# Autodesk Inventor assembly: 0005-00-00 Ansamblu_General_V1
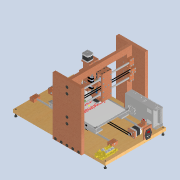
[picture p0: Inventor's stored thumbnail of the model, 180x180]
Saved by Autodesk Inventor 2020 (Build 240168000, 168)
## iProperties
Created: 2020-12-26
Part Number: 0005-00-00 Ansamblu_General_V1
Document SubType Name: Assembly
Designer: Iulian Bors
Author: Iulian Bors
## Documents named in this file (14)
- Z:\I.A.B\Proiecte\0005 I.A.B 3d 2.0 Imprimanta aracet\0005-00-00 Ansamblu_General_V1.iam
- Z:\I.A.B\Proiecte\0005 I.A.B 3d 2.0 Imprimanta aracet\10 Mecanic\0005-10-01 Cadru.iam
- Z:\I.A.B\Proiecte\0005 I.A.B 3d 2.0 Imprimanta aracet\10 Mecanic\0005-10-02 X axis.iam
- Z:\I.A.B\Proiecte\0005 I.A.B 3d 2.0 Imprimanta aracet\10 Mecanic\0005-10-03 Y axis.iam
- Z:\I.A.B\Proiecte\0005 I.A.B 3d 2.0 Imprimanta aracet\10 Mecanic\0005-10-04 Z axis and extruder.iam
- Z:\I.A.B\Proiecte\0005 I.A.B 3d 2.0 Imprimanta aracet\20 Electric\0005-20-01 Assembly Arduino Mega RAMPS 1.4.iam
- Z:\I.A.B\Proiecte\0005 I.A.B 3d 2.0 Imprimanta aracet\20 Electric\Inlet Module Plug Fuse Switch Male Power Socket 10A 250V 3 Pin IEC320 C14.ipt
- Z:\I.A.B\Proiecte\0005 I.A.B 3d 2.0 Imprimanta aracet\20 Electric\00005-20-1004 PowerSupplyLedMax500.ipt
- Z:\I.A.B\Proiecte\0005 I.A.B 3d 2.0 Imprimanta aracet\10 Mecanic\0005-10-1044 DIN EN ISO 1483 - ST3.5 x 13 - C.ipt
- Z:\I.A.B\Proiecte\0005 I.A.B 3d 2.0 Imprimanta aracet\20 Electric\0005-20-1003 Switch.ipt
- Z:\I.A.B\Proiecte\0005 I.A.B 3d 2.0 Imprimanta aracet\10 Mecanic\0005-10-028 suport senzor y.ipt
- Z:\I.A.B\Proiecte\0005 I.A.B 3d 2.0 Imprimanta aracet\10 Mecanic\0005-10-1032.ipt
- Z:\I.A.B\Proiecte\0005 I.A.B 3d 2.0 Imprimanta aracet\10 Mecanic\0005-10-1019 ISO 4762 - M3 x 30ISO.ipt
- Z:\I.A.B\Proiecte\0005 I.A.B 3d 2.0 Imprimanta aracet\10 Mecanic\0005-10-030 Activator senzor x.ipt
## Components (23 placed, 13 different names)
1. 0005-10-01 Cadru:1 [sub-assembly] — Insert:1, Mate:1, Mate:3, Flush:1, Flush:2, Mate:4, Flush:3, Flush:4, Mate:5, Mate:6, Mate:7, Mate:9, Mate:12, Mate:16, Mate:17, Insert:18, Insert:19, Mate:19, Flush:11
2. 0005-10-02 X axis:1 [sub-assembly] — Insert:1, Mate:1, Insert:2, Insert:3, Mate:18, Flush:10
3. 0005-10-03 Y axis:1 [sub-assembly] — Mate:3, Flush:1, Flush:2, Mate:11, Flush:5, Mate:13, Flush:6
4. 0005-10-04 Z axis and extruder:1 [sub-assembly] — Insert:2, Insert:3, Mate:15, Flush:8, Flush:9
5. 0005-20-01 Assembly Arduino Mega RAMPS 1.4:1 [sub-assembly] — Mate:4, Flush:3, Flush:4, Insert:15, Insert:16, Insert:17
6. Inlet Module Plug Fuse Switch Male Power Socket 10A 250V 3 Pin IEC320 C14:1 — Mate:5, Mate:6, Mate:7, Insert:4, Insert:5
7. 00005-20-1004 PowerSupplyLedMax500:1 — Mate:9, Mate:16, Mate:17
8. DIN EN ISO 1483 - C ST3.5 x 13 - C:1 — Insert:4
9. DIN EN ISO 1483 - C ST3.5 x 13 - C:2 — Insert:5
10. 0005-20-1003 Switch:1 — Mate:11, Mate:12, Flush:5, Insert:13, Insert:14
11. 0005-20-1003 Switch:2 — Mate:15, Flush:8, Flush:9, Insert:11, Insert:12
12. 0005-20-1003 Switch:3 — Mate:18, Flush:10
13. 0005-10-028 suport senzor y:1 — Mate:13, Flush:6
14. DIN 7984 M3 x 16:1 — Insert:14
15. DIN 7984 M3 x 16:2 — Insert:13
16. DIN 7984 M3 x 16:3 — Insert:12
17. DIN 7984 M3 x 16:4 — Insert:11
18. ISO 4762 M3 x 30:1 — Insert:15
19. ISO 4762 M3 x 30:2 — Insert:17
20. ISO 4762 M3 x 30:3 — Insert:16
21. ISO 4762 M3 x 30:4 — Insert:18
22. ISO 4762 M3 x 30:5 — Insert:19
23. 0005-10-030 Activator senzor x:1 — Mate:19, Flush:11
## Relationships (39: Mate 15, Insert 14, Flush 10)
- Insert:1: 0005-10-01 Cadru:1 ↔ 0005-10-02 X axis:1
- Mate:1: 0005-10-01 Cadru:1 ↔ 0005-10-02 X axis:1
- Mate:3: 0005-10-01 Cadru:1 ↔ 0005-10-03 Y axis:1
- Flush:1 (110 mm): 0005-10-01 Cadru:1 ↔ 0005-10-03 Y axis:1
- Flush:2 (5.193 mm): 0005-10-01 Cadru:1 ↔ 0005-10-03 Y axis:1
- Insert:2: 0005-10-02 X axis:1 ↔ 0005-10-04 Z axis and extruder:1
- Insert:3: 0005-10-02 X axis:1 ↔ 0005-10-04 Z axis and extruder:1
- Mate:4 (3 mm): 0005-10-01 Cadru:1 ↔ 0005-20-01 Assembly Arduino Mega RAMPS 1.4:1
- Flush:3 (-10 mm): 0005-10-01 Cadru:1 ↔ 0005-20-01 Assembly Arduino Mega RAMPS 1.4:1
- Flush:4 (20 mm): 0005-10-01 Cadru:1 ↔ 0005-20-01 Assembly Arduino Mega RAMPS 1.4:1
- Mate:5: 0005-10-01 Cadru:1 ↔ Inlet Module Plug Fuse Switch Male Power Socket 10A 250V 3 Pin IEC320 C14:1
- Mate:6: 0005-10-01 Cadru:1 ↔ Inlet Module Plug Fuse Switch Male Power Socket 10A 250V 3 Pin IEC320 C14:1
- Mate:7 (2 mm): 0005-10-01 Cadru:1 ↔ Inlet Module Plug Fuse Switch Male Power Socket 10A 250V 3 Pin IEC320 C14:1
- Mate:9: 0005-10-01 Cadru:1 ↔ 00005-20-1004 PowerSupplyLedMax500:1
- Insert:4: Inlet Module Plug Fuse Switch Male Power Socket 10A 250V 3 Pin IEC320 C14:1 ↔ DIN EN ISO 1483 - C ST3.5 x 13 - C:1
- Insert:5: Inlet Module Plug Fuse Switch Male Power Socket 10A 250V 3 Pin IEC320 C14:1 ↔ DIN EN ISO 1483 - C ST3.5 x 13 - C:2
- Mate:11 (8 mm): 0005-10-03 Y axis:1 ↔ 0005-20-1003 Switch:1
- Mate:12: 0005-10-01 Cadru:1 ↔ 0005-20-1003 Switch:1
- Flush:5: 0005-10-03 Y axis:1 ↔ 0005-20-1003 Switch:1
- Mate:13: 0005-10-03 Y axis:1 ↔ 0005-10-028 suport senzor y:1
- Flush:6: 0005-10-03 Y axis:1 ↔ 0005-10-028 suport senzor y:1
- Mate:15: 0005-10-04 Z axis and extruder:1 ↔ 0005-20-1003 Switch:2
- Flush:8: 0005-10-04 Z axis and extruder:1 ↔ 0005-20-1003 Switch:2
- Flush:9: 0005-10-04 Z axis and extruder:1 ↔ 0005-20-1003 Switch:2
- Insert:11: 0005-20-1003 Switch:2 ↔ DIN 7984 M3 x 16:4
- Insert:12: 0005-20-1003 Switch:2 ↔ DIN 7984 M3 x 16:3
- Insert:13: 0005-20-1003 Switch:1 ↔ DIN 7984 M3 x 16:2
- Insert:14: 0005-20-1003 Switch:1 ↔ DIN 7984 M3 x 16:1
- Insert:15: 0005-20-01 Assembly Arduino Mega RAMPS 1.4:1 ↔ ISO 4762 M3 x 30:1
- Insert:16: 0005-20-01 Assembly Arduino Mega RAMPS 1.4:1 ↔ ISO 4762 M3 x 30:3
- Insert:17: 0005-20-01 Assembly Arduino Mega RAMPS 1.4:1 ↔ ISO 4762 M3 x 30:2
- Mate:16: 0005-10-01 Cadru:1 ↔ 00005-20-1004 PowerSupplyLedMax500:1
- Mate:17: 0005-10-01 Cadru:1 ↔ 00005-20-1004 PowerSupplyLedMax500:1
- Insert:18: 0005-10-01 Cadru:1 ↔ ISO 4762 M3 x 30:4
- Insert:19: 0005-10-01 Cadru:1 ↔ ISO 4762 M3 x 30:5
- Mate:18: 0005-10-02 X axis:1 ↔ 0005-20-1003 Switch:3
- Flush:10: 0005-10-02 X axis:1 ↔ 0005-20-1003 Switch:3
- Mate:19: 0005-10-01 Cadru:1 ↔ 0005-10-030 Activator senzor x:1
- Flush:11: 0005-10-01 Cadru:1 ↔ 0005-10-030 Activator senzor x:1
